# Autodesk Inventor assembly: arm
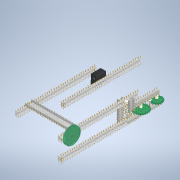
[picture p0: Inventor's stored thumbnail of the model, 180x180]
Saved by Autodesk Inventor 2020 (Build 240168000, 168)
## iProperties
Created: 2019-10-24
Part Number: arm
Document SubType Name: Assembly
Designer: Alex Zaccardelli
Author: Alex Zaccardelli
## Documents named in this file (16)
- D:\TrayBot Project\arm.iam
- D:\TrayBot Project\SIGBotsCADLibrary-20191023T040826Z-001\SIGBotsCADLibrary\SIGBotsCADLibrary\Structure\C-Channel 2 x 35 (aluminum).ipt
- D:\TrayBot Project\SIGBotsCADLibrary-20191023T040826Z-001\SIGBotsCADLibrary\SIGBotsCADLibrary\Motion\Gear HS 84 tooth (fixed).iam
- D:\TrayBot Project\SIGBotsCADLibrary-20191023T040826Z-001\SIGBotsCADLibrary\SIGBotsCADLibrary\Motion\Spacer 1.0 unit.ipt
- D:\TrayBot Project\SIGBotsCADLibrary-20191023T040826Z-001\SIGBotsCADLibrary\SIGBotsCADLibrary\Motion\Spacer 0.25 unit.ipt
- D:\TrayBot Project\SIGBotsCADLibrary-20191023T040826Z-001\SIGBotsCADLibrary\SIGBotsCADLibrary\Structure\C-Channel 3 x 16 (aluminum).ipt
- D:\TrayBot Project\SIGBotsCADLibrary-20191023T040826Z-001\SIGBotsCADLibrary\SIGBotsCADLibrary\Motion\Lock Plate.ipt
- D:\TrayBot Project\SIGBotsCADLibrary-20191023T040826Z-001\SIGBotsCADLibrary\SIGBotsCADLibrary\Structure\C-Channel 2 x 5 (aluminum).ipt
- D:\TrayBot Project\SIGBotsCADLibrary-20191023T040826Z-001\SIGBotsCADLibrary\SIGBotsCADLibrary\Structure\Plate 2 x 5 (aluminum).ipt
- D:\TrayBot Project\SIGBotsCADLibrary-20191023T040826Z-001\SIGBotsCADLibrary\SIGBotsCADLibrary\Motion\Spacer 0.50 unit.ipt
- D:\TrayBot Project\SIGBotsCADLibrary-20191023T040826Z-001\SIGBotsCADLibrary\SIGBotsCADLibrary\Structure\C-Channel 2 x 15 (aluminum).ipt
- D:\TrayBot Project\SIGBotsCADLibrary-20191023T040826Z-001\SIGBotsCADLibrary\SIGBotsCADLibrary\V5_Smart_Motor_276-4840 (1).ipt
- D:\TrayBot Project\SIGBotsCADLibrary-20191023T040826Z-001\SIGBotsCADLibrary\SIGBotsCADLibrary\Motion\Sprocket HS 24 tooth.ipt
- D:\TrayBot Project\SIGBotsCADLibrary-20191023T040826Z-001\SIGBotsCADLibrary\SIGBotsCADLibrary\Motion\Sprocket HS 18 tooth.ipt
- D:\TrayBot Project\SIGBotsCADLibrary-20191023T040826Z-001\SIGBotsCADLibrary\SIGBotsCADLibrary\Structure\Standoff 1.0 inch.ipt
- D:\TrayBot Project\SIGBotsCADLibrary-20191023T040826Z-001\SIGBotsCADLibrary\SIGBotsCADLibrary\Structure\C-Channel 2 x 10 (aluminum).ipt
## Components (42 placed, 15 different names)
1. C-Channel 2 x 35 (aluminum):1 — Mate:3, Mate:4, Mate:8, Mate:11, Mate:12, Mate:16, Mate:17, Mate:18, Mate:22, Mate:23, Mate:24, Mate:25, Mate:26, Mate:27, Mate:28, Mate:29, Mate:30, Mate:31, Mate:35, Mate:36, Mate:37, Angle:1, Mate:91, Mate:92, Mate:93, Mate:95
2. Gear HS 84 tooth (fixed):1 [sub-assembly] — Mate:13, Mate:14, Mate:15
3. Spacer 1.0 unit:1 — Mate:1, Mate:2, Mate:3, Mate:4
4. Spacer 0.25 unit:1 — Mate:1, Mate:2, Mate:15
5. Spacer 1.0 unit:2 — Mate:8, Mate:13, Mate:14
6. Spacer 1.0 unit:3 — Mate:12
7. Spacer 0.25 unit:3 — Mate:11
8. C-Channel 3 x 16 (aluminum):1 — Mate:16, Mate:17, Mate:18, Mate:19, Mate:20, Mate:21
9. C-Channel 2 x 35 (aluminum):2 — Mate:19, Mate:20, Mate:21
10. Lock Plate:1 — Mate:22, Mate:23, Mate:24
11. Lock Plate:2 — Mate:25, Mate:26, Mate:27
12. Spacer 1.0 unit:4 — Mate:28, Mate:29, Mate:40, Mate:41
13. Spacer 1.0 unit:5 — Mate:30, Mate:31, Mate:38, Mate:39
14. Plate 3 x 4:1 — Mate:35, Mate:36, Mate:37, Mate:45, Mate:46
15. C-Channel 2 x 5 (aluminum):1 — Mate:42, Mate:43, Mate:44, Mate:55
16. Spacer 0.50 unit:1 — Mate:38, Mate:39, Mate:42
17. Spacer 0.50 unit:2 — Mate:40, Mate:41, Mate:43, Mate:44
18. Spacer 0.25 unit:4 — Mate:45, Mate:46, Mate:47, Mate:48
19. Spacer 0.25 unit:5 — Mate:47, Mate:48, Mate:49, Mate:50
20. Spacer 0.25 unit:6 — Mate:49, Mate:50, Mate:51, Mate:52, Mate:56
21. C-Channel 2 x 15 (aluminum):1 — Mate:53, Mate:54, Mate:60, Mate:61, Mate:68, Mate:69, Mate:82, Mate:89, Mate:90, Angle:1
22. Spacer 0.25 unit:7 — Mate:51, Mate:52, Mate:53, Mate:54
23. Spacer 0.50 unit:3 — Mate:55, Mate:56
24. Spacer 1.0 unit:6 — Mate:60, Mate:61, Mate:62, Mate:63
25. Sprocket HS 24 tooth:1 — Mate:64, Mate:65, Mate:74
26. Spacer 0.50 unit:4 — Mate:62, Mate:63, Mate:64, Mate:65
27. Spacer 1.0 unit:7 — Mate:68, Mate:69
28. Spacer 0.50 unit:5 — Mate:70, Mate:71
29. Sprocket HS 18 tooth:1 — Mate:70, Mate:71, Mate:72, Mate:73
30. C-Channel 2 x 15 (aluminum):2 — Mate:72, Mate:73, Mate:74, Mate:81
31. Spacer 0.25 unit:8 — Mate:79, Mate:80
32. Spacer 0.25 unit:9
33. Spacer 0.25 unit:10 — Mate:82
34. Standoff 1.0 inch:1 — Mate:79, Mate:80, Mate:81
35. Spacer 0.25 unit:11
36. Spacer 0.25 unit:12
37. Spacer 0.25 unit:13 — Mate:89, Mate:90
38. Standoff 1.0 inch:2
39. V5_Smart_Motor_276-4840 (1):1
40. C-Channel 2 x 35 (aluminum):3
41. C-Channel 2 x 10 (aluminum):1 — Mate:91, Mate:92, Mate:93, Mate:94, Mate:96, Mate:97
42. C-Channel 2 x 35 (aluminum):4 — Mate:94, Mate:95, Mate:96, Mate:97
## Relationships (89: Mate 88, Angle 1)
- Mate:1: Spacer 1.0 unit:1 ↔ Spacer 0.25 unit:1
- Mate:2: Spacer 1.0 unit:1 ↔ Spacer 0.25 unit:1
- Mate:3: C-Channel 2 x 35 (aluminum):1 ↔ Spacer 1.0 unit:1
- Mate:4: C-Channel 2 x 35 (aluminum):1 ↔ Spacer 1.0 unit:1
- Mate:8: C-Channel 2 x 35 (aluminum):1 ↔ Spacer 1.0 unit:2
- [Mate]: Spacer 1.0 unit:3 ↔ Spacer 0.25 unit:3
- [Mate]: Spacer 1.0 unit:3 ↔ Spacer 0.25 unit:3
- Mate:11: C-Channel 2 x 35 (aluminum):1 ↔ Spacer 0.25 unit:3
- Mate:12: C-Channel 2 x 35 (aluminum):1 ↔ Spacer 1.0 unit:3
- Mate:13: Gear HS 84 tooth (fixed):1 ↔ Spacer 1.0 unit:2
- Mate:14: Gear HS 84 tooth (fixed):1 ↔ Spacer 1.0 unit:2
- Mate:15: Gear HS 84 tooth (fixed):1 ↔ Spacer 0.25 unit:1
- Mate:16: C-Channel 2 x 35 (aluminum):1 ↔ C-Channel 3 x 16 (aluminum):1
- Mate:17: C-Channel 2 x 35 (aluminum):1 ↔ C-Channel 3 x 16 (aluminum):1
- Mate:18: C-Channel 2 x 35 (aluminum):1 ↔ C-Channel 3 x 16 (aluminum):1
- Mate:19: C-Channel 3 x 16 (aluminum):1 ↔ C-Channel 2 x 35 (aluminum):2
- Mate:20: C-Channel 3 x 16 (aluminum):1 ↔ C-Channel 2 x 35 (aluminum):2
- Mate:21: C-Channel 3 x 16 (aluminum):1 ↔ C-Channel 2 x 35 (aluminum):2
- Mate:22: C-Channel 2 x 35 (aluminum):1 ↔ Lock Plate:1
- Mate:23: C-Channel 2 x 35 (aluminum):1 ↔ Lock Plate:1
- Mate:24: C-Channel 2 x 35 (aluminum):1 ↔ Lock Plate:1
- Mate:25: C-Channel 2 x 35 (aluminum):1 ↔ Lock Plate:2
- Mate:26: C-Channel 2 x 35 (aluminum):1 ↔ Lock Plate:2
- Mate:27: C-Channel 2 x 35 (aluminum):1 ↔ Lock Plate:2
- Mate:28: C-Channel 2 x 35 (aluminum):1 ↔ Spacer 1.0 unit:4
- Mate:29: C-Channel 2 x 35 (aluminum):1 ↔ Spacer 1.0 unit:4
- Mate:30: C-Channel 2 x 35 (aluminum):1 ↔ Spacer 1.0 unit:5
- Mate:31: C-Channel 2 x 35 (aluminum):1 ↔ Spacer 1.0 unit:5
- Mate:35: C-Channel 2 x 35 (aluminum):1 ↔ Plate 3 x 4:1
- Mate:36: C-Channel 2 x 35 (aluminum):1 ↔ Plate 3 x 4:1
- Mate:37: C-Channel 2 x 35 (aluminum):1 ↔ Plate 3 x 4:1
- Mate:38: Spacer 1.0 unit:5 ↔ Spacer 0.50 unit:1
- Mate:39: Spacer 1.0 unit:5 ↔ Spacer 0.50 unit:1
- Mate:40: Spacer 1.0 unit:4 ↔ Spacer 0.50 unit:2
- Mate:41: Spacer 1.0 unit:4 ↔ Spacer 0.50 unit:2
- Mate:42: C-Channel 2 x 5 (aluminum):1 ↔ Spacer 0.50 unit:1
- Mate:43: C-Channel 2 x 5 (aluminum):1 ↔ Spacer 0.50 unit:2
- Mate:44: C-Channel 2 x 5 (aluminum):1 ↔ Spacer 0.50 unit:2
- Mate:45: Plate 3 x 4:1 ↔ Spacer 0.25 unit:4
- Mate:46: Plate 3 x 4:1 ↔ Spacer 0.25 unit:4
- Mate:47: Spacer 0.25 unit:4 ↔ Spacer 0.25 unit:5
- Mate:48: Spacer 0.25 unit:4 ↔ Spacer 0.25 unit:5
- Mate:49: Spacer 0.25 unit:5 ↔ Spacer 0.25 unit:6
- Mate:50: Spacer 0.25 unit:5 ↔ Spacer 0.25 unit:6
- Mate:51: Spacer 0.25 unit:6 ↔ Spacer 0.25 unit:7
- Mate:52: Spacer 0.25 unit:6 ↔ Spacer 0.25 unit:7
- Mate:53: C-Channel 2 x 15 (aluminum):1 ↔ Spacer 0.25 unit:7
- Mate:54: C-Channel 2 x 15 (aluminum):1 ↔ Spacer 0.25 unit:7
- Mate:55: C-Channel 2 x 5 (aluminum):1 ↔ Spacer 0.50 unit:3
- Mate:56: Spacer 0.25 unit:6 ↔ Spacer 0.50 unit:3
- Mate:60: C-Channel 2 x 15 (aluminum):1 ↔ Spacer 1.0 unit:6
- Mate:61: C-Channel 2 x 15 (aluminum):1 ↔ Spacer 1.0 unit:6
- Mate:62: Spacer 1.0 unit:6 ↔ Spacer 0.50 unit:4
- Mate:63: Spacer 1.0 unit:6 ↔ Spacer 0.50 unit:4
- Mate:64: Sprocket HS 24 tooth:1 ↔ Spacer 0.50 unit:4
- Mate:65: Sprocket HS 24 tooth:1 ↔ Spacer 0.50 unit:4
- [Mate]: Spacer 1.0 unit:7 ↔ Spacer 0.50 unit:5
- [Mate]: Spacer 1.0 unit:7 ↔ Spacer 0.50 unit:5
- Mate:68: C-Channel 2 x 15 (aluminum):1 ↔ Spacer 1.0 unit:7
- Mate:69: C-Channel 2 x 15 (aluminum):1 ↔ Spacer 1.0 unit:7
- Mate:70: Spacer 0.50 unit:5 ↔ Sprocket HS 18 tooth:1
- Mate:71: Spacer 0.50 unit:5 ↔ Sprocket HS 18 tooth:1
- Mate:72: Sprocket HS 18 tooth:1 ↔ C-Channel 2 x 15 (aluminum):2
- Mate:73: Sprocket HS 18 tooth:1 ↔ C-Channel 2 x 15 (aluminum):2
- Mate:74: Sprocket HS 24 tooth:1 ↔ C-Channel 2 x 15 (aluminum):2
- [Mate]: Spacer 0.25 unit:8 ↔ Spacer 0.25 unit:9
- [Mate]: Spacer 0.25 unit:8 ↔ Spacer 0.25 unit:9
- [Mate]: Spacer 0.25 unit:9 ↔ Spacer 0.25 unit:10
- [Mate]: Spacer 0.25 unit:9 ↔ Spacer 0.25 unit:10
- Mate:79: Spacer 0.25 unit:8 ↔ Standoff 1.0 inch:1
- Mate:80: Spacer 0.25 unit:8 ↔ Standoff 1.0 inch:1
- Mate:81: C-Channel 2 x 15 (aluminum):2 ↔ Standoff 1.0 inch:1
- Mate:82: C-Channel 2 x 15 (aluminum):1 ↔ Spacer 0.25 unit:10
- [Mate]: Spacer 0.25 unit:11 ↔ Spacer 0.25 unit:12
- [Mate]: Spacer 0.25 unit:11 ↔ Spacer 0.25 unit:12
- [Mate]: Spacer 0.25 unit:12 ↔ Spacer 0.25 unit:13
- [Mate]: Spacer 0.25 unit:12 ↔ Spacer 0.25 unit:13
- [Mate]: Spacer 0.25 unit:11 ↔ Standoff 1.0 inch:2
- [Mate]: Spacer 0.25 unit:11 ↔ Standoff 1.0 inch:2
- Mate:89: C-Channel 2 x 15 (aluminum):1 ↔ Spacer 0.25 unit:13
- Mate:90: C-Channel 2 x 15 (aluminum):1 ↔ Spacer 0.25 unit:13
- Angle:1 (0 deg): C-Channel 2 x 35 (aluminum):1 ↔ C-Channel 2 x 15 (aluminum):1
- Mate:91: C-Channel 2 x 35 (aluminum):1 ↔ C-Channel 2 x 10 (aluminum):1
- Mate:92: C-Channel 2 x 35 (aluminum):1 ↔ C-Channel 2 x 10 (aluminum):1
- Mate:93: C-Channel 2 x 35 (aluminum):1 ↔ C-Channel 2 x 10 (aluminum):1
- Mate:94: C-Channel 2 x 10 (aluminum):1 ↔ C-Channel 2 x 35 (aluminum):4
- Mate:95: C-Channel 2 x 35 (aluminum):1 ↔ C-Channel 2 x 35 (aluminum):4
- Mate:96: C-Channel 2 x 10 (aluminum):1 ↔ C-Channel 2 x 35 (aluminum):4
- Mate:97: C-Channel 2 x 10 (aluminum):1 ↔ C-Channel 2 x 35 (aluminum):4
## Named parameters: d8_d0 = 0 mm, d9_d1 = 0 mm, d75_d71 = 0 mm, d76_d72 = 0 mm, d108_d48 = 0 mm, d109_d49 = 0 mm, d110_d50 = 0 mm, d111_d51 = 0 mm, d116_d108_d48 = 0 mm, d117_d109_d49 = 0 mm, d118_d110_d50 = 0 mm, d119_d111_d51 = 0 mm, d120_d112 = 0 mm, d121_d113 = 0 mm
